# Autodesk Inventor assembly: plugassmbly
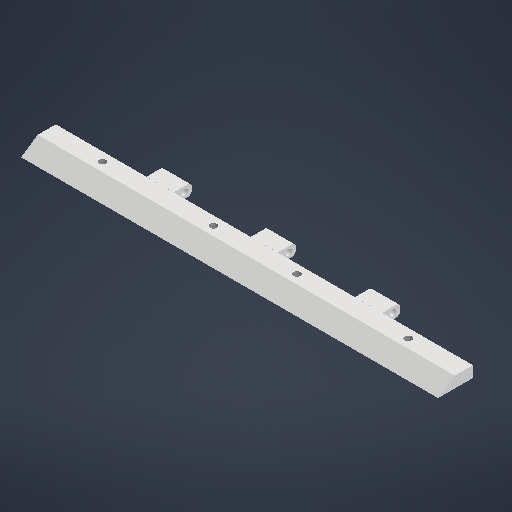
[picture p0: Inventor's stored thumbnail of the model, 512x512]
Saved by Autodesk Inventor 2026.2 (Build 302298010, 298A)
## iProperties
Created: 2026-05-09
Part Number: plugassmbly
Document SubType Name: Assembly
Designer: karol
Author: karol
## Documents named in this file (3)
- C:\Users\karol\Desktop\BOLT\cad\assembly\plugassmbly.iam
- C:\Users\karol\Desktop\BOLT\cad\ready parts\pługmoj.ipt
- C:\Users\karol\Desktop\BOLT\cad\ready parts\mocowanie do pługu.ipt
## Components (2 placed, 2 different names)
1. mocowanie do pługu:1 — Zestawiające:1, Zestawiające:2
2. pługmoj:1 — Zestawiające:1, Zestawiające:2
## Relationships (2: Mate 2)
- Zestawiające:1 [Mate]: mocowanie do pługu:1 ↔ pługmoj:1
- Zestawiające:2 [Mate]: mocowanie do pługu:1 ↔ pługmoj:1
